# Autodesk Inventor assembly: Joes_Robot
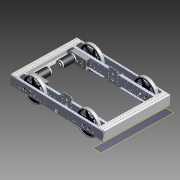
[picture p0: Inventor's stored thumbnail of the model, 180x180]
Saved by Autodesk Inventor 2015 SP1 (Build 190203100, 203)
## iProperties
Created: 2015-01-23
Part Number: Joes_Robot
Document SubType Name: Assembly
Designer: 55221
Author: 55221
## Documents named in this file (8)
- Z:\RoboEaglesCAD\2015CAD\Misc\Joes_Robot.iam
- Z:\RoboEaglesCAD\2015CAD\wheelBase\Outside Sheet Square.ipt
- Z:\RoboEaglesCAD\2015CAD\wheelBase\Inside Sheet Square.ipt
- Z:\RoboEaglesCAD\2015CAD\wheelBase\TB Output Shaft Hex L-Base 2.ipt
- Z:\RoboEaglesCAD\2015CAD\actualWheelBase\Drive Base\Parts\Imported Components\Sheet Metal Front-Back\Sheet Metal Front-Back.ipt
- Z:\RoboEaglesCAD\2015CAD\actualWheelBase\Drive Base\Parts\simpleGBFull.iam
- Z:\RoboEaglesCAD\2015CAD\actualWheelBase\Drive Base\Parts\8inDriveWheel.iam
- Z:\RoboEaglesCAD\2015CAD\wheelBase\Hex Bearing.ipt
## Components (18 placed, 7 different names)
1. Outside Sheet Square:1 — Mate:181, Mate:183, Mate:189, Mate:206, Mate:207, Insert:14, Insert:18
2. Inside Sheet Square:1 — Mate:150, Mate:182, Mate:184, Mate:188, Mate:204, Mate:205, Angle:9, Insert:15, Insert:19, Insert:20
3. Inside Sheet Square:2 — Mate:180, Mate:185, Insert:1, Angle:5, Mate:201, Mate:202, Mate:203, Insert:16, Insert:21
4. Outside Sheet Square:2 — Mate:178, Mate:179, Mate:186, Mate:187, Mate:208, Mate:209, Mate:263, Insert:17, Insert:22
5. TB Output Shaft Hex L-Base 2:3 — Mate:150, Angle:8
6. Sheet Metal Front-Back:1 — Mate:178, Mate:179, Mate:180, Mate:181, Mate:182, Mate:183, Mate:184, Flush:22
7. Sheet Metal Front-Back:2 — Mate:185, Mate:186, Mate:187, Mate:188, Mate:189, Mate:263
8. simpleGBFull:1 [sub-assembly] — Angle:9
9. 8inDriveWheel:1 [sub-assembly]
10. simpleGBFull:2 [sub-assembly] — Insert:1, Angle:5, Mate:198, Mate:199
11. TB Output Shaft Hex L-Base 2:4 — Mate:198, Mate:199, Mate:200, Angle:6, Angle:7
12. 8inDriveWheel:4 [sub-assembly] — Mate:200, Angle:6, Mate:201
13. 8inDriveWheel:5 [sub-assembly] — Mate:202, Mate:203
14. 8inDriveWheel:6 [sub-assembly] — Mate:204, Mate:205
15. Hex Bearing:1 — Mate:206, Mate:207, Angle:8
16. Hex Bearing:2 — Mate:208, Mate:209, Angle:7
17. Sheet Metal Front-Back:1 — Insert:14, Insert:15, Insert:16, Insert:17
18. Sheet Metal Front-Back:2 — Insert:18, Insert:19, Insert:20, Insert:21, Insert:22
## Relationships (48: Mate 32, Insert 10, Angle 5, Flush 1)
- [Mate]: TB Output Shaft Hex L-Base 2:3 ↔ simpleGBFull:1
- [Mate]: Inside Sheet Square:1 ↔ simpleGBFull:1
- Mate:150: Inside Sheet Square:1 ↔ TB Output Shaft Hex L-Base 2:3
- [Mate]: TB Output Shaft Hex L-Base 2:3 ↔ simpleGBFull:1
- Mate:178: Outside Sheet Square:2 ↔ Sheet Metal Front-Back:1
- Mate:179: Outside Sheet Square:2 ↔ Sheet Metal Front-Back:1
- Mate:180: Inside Sheet Square:2 ↔ Sheet Metal Front-Back:1
- Mate:181: Outside Sheet Square:1 ↔ Sheet Metal Front-Back:1
- Mate:182: Inside Sheet Square:1 ↔ Sheet Metal Front-Back:1
- Mate:183: Outside Sheet Square:1 ↔ Sheet Metal Front-Back:1
- Mate:184: Inside Sheet Square:1 ↔ Sheet Metal Front-Back:1
- Mate:185: Inside Sheet Square:2 ↔ Sheet Metal Front-Back:2
- Mate:186: Outside Sheet Square:2 ↔ Sheet Metal Front-Back:2
- Mate:187: Outside Sheet Square:2 ↔ Sheet Metal Front-Back:2
- Mate:188: Inside Sheet Square:1 ↔ Sheet Metal Front-Back:2
- Mate:189: Outside Sheet Square:1 ↔ Sheet Metal Front-Back:2
- [Mate]: TB Output Shaft Hex L-Base 2:3 ↔ 8inDriveWheel:1
- [Mate]: TB Output Shaft Hex L-Base 2:3 ↔ 8inDriveWheel:1
- [Mate]: Inside Sheet Square:1 ↔ 8inDriveWheel:1
- Insert:1: Inside Sheet Square:2 ↔ simpleGBFull:2
- Angle:5 (0 deg): Inside Sheet Square:2 ↔ simpleGBFull:2
- Mate:198: simpleGBFull:2 ↔ TB Output Shaft Hex L-Base 2:4
- Mate:199: simpleGBFull:2 ↔ TB Output Shaft Hex L-Base 2:4
- Mate:200: TB Output Shaft Hex L-Base 2:4 ↔ 8inDriveWheel:4
- Angle:6 (0 deg): TB Output Shaft Hex L-Base 2:4 ↔ 8inDriveWheel:4
- Mate:201: Inside Sheet Square:2 ↔ 8inDriveWheel:4
- Mate:202: Inside Sheet Square:2 ↔ 8inDriveWheel:5
- Mate:203: Inside Sheet Square:2 ↔ 8inDriveWheel:5
- Mate:204: Inside Sheet Square:1 ↔ 8inDriveWheel:6
- Mate:205: Inside Sheet Square:1 ↔ 8inDriveWheel:6
- Mate:206: Outside Sheet Square:1 ↔ Hex Bearing:1
- Mate:207: Outside Sheet Square:1 ↔ Hex Bearing:1
- Mate:208: Outside Sheet Square:2 ↔ Hex Bearing:2
- Mate:209: Outside Sheet Square:2 ↔ Hex Bearing:2
- Angle:7 (0 deg): TB Output Shaft Hex L-Base 2:4 ↔ Hex Bearing:2
- Angle:8 (0 deg): TB Output Shaft Hex L-Base 2:3 ↔ Hex Bearing:1
- Angle:9 (0 deg): Inside Sheet Square:1 ↔ simpleGBFull:1
- Mate:263: Outside Sheet Square:2 ↔ Sheet Metal Front-Back:2
- Flush:22 (63.5 mm): Sheet Metal Front-Back:1
- Insert:14: Outside Sheet Square:1 ↔ Sheet Metal Front-Back:1
- Insert:15: Inside Sheet Square:1 ↔ Sheet Metal Front-Back:1
- Insert:16: Inside Sheet Square:2 ↔ Sheet Metal Front-Back:1
- Insert:17: Outside Sheet Square:2 ↔ Sheet Metal Front-Back:1
- Insert:18: Outside Sheet Square:1 ↔ Sheet Metal Front-Back:2
- Insert:19: Inside Sheet Square:1 ↔ Sheet Metal Front-Back:2
- Insert:20: Inside Sheet Square:1 ↔ Sheet Metal Front-Back:2
- Insert:21: Inside Sheet Square:2 ↔ Sheet Metal Front-Back:2
- Insert:22: Outside Sheet Square:2 ↔ Sheet Metal Front-Back:2
